# Autodesk Inventor assembly: inner
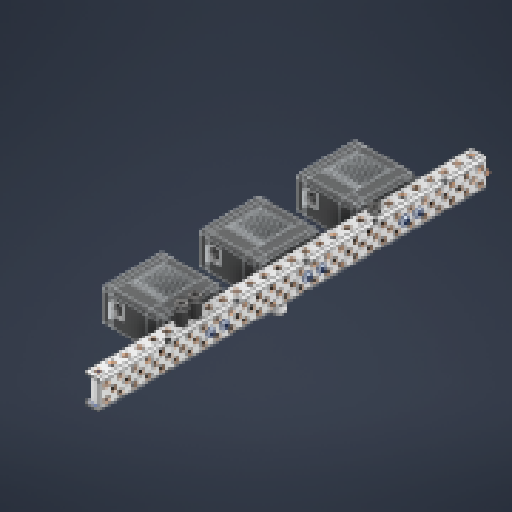
[picture p0: Inventor's stored thumbnail of the model, 512x512]
Saved by Autodesk Inventor 2024 (Build 280153000, 153)
## iProperties
Created: 2023-10-29
Part Number: inner
Document SubType Name: Assembly
Designer: avere
Author: avere
## Documents named in this file (17)
- C:\Users\avere\Documents\rbp_cad\zoomba_v0.1\chassis\drivebay\inner.iam
- C:\Users\avere\Documents\rbp_cad\VEX-CAD-Inventor-1.41\Structure\C Channel\Aluminum 1x2x1\Alu C 1x2x1x28.ipt
- C:\Users\avere\Documents\rbp_cad\VEX-CAD-Inventor-1.41\Electronics\Motors with Screws\SteelM-StarS.iam
- C:\Users\avere\Documents\rbp_cad\VEX-CAD-Inventor-1.41\Electronics\Motors with Screws.iam
- C:\Users\avere\Documents\rbp_cad\hardware\.375 OD Aluminum Spacer 0.875.ipt
- C:\Users\avere\Documents\rbp_cad\VEX-CAD-Inventor-1.41\Motion\Spacers\Spacer Nylon .375 OD.ipt
- C:\Users\avere\Documents\rbp_cad\VEX-CAD-Inventor-1.41\Motion\Spacers\Spacer Nylon .375 OD\NSpacer .375 OD x .500.ipt
- C:\Users\avere\Documents\rbp_cad\zoomba_v0.1\chassis\drivebay\custom_parts\washer_thick.ipt
- C:\Users\avere\Documents\rbp_cad\VEX-CAD-Inventor-1.41\Motion\Spacers\Spacer Nylon .500 OD\NSpacer White .500 OD x .250.ipt
- C:\Users\avere\Documents\rbp_cad\VEX-CAD-Inventor-1.41\Motion\Spacers\Spacer Nylon .500 OD.ipt
- C:\Users\avere\Documents\rbp_cad\VEX-CAD-Inventor-1.41\Structure\Standoff\Standoff .875.ipt
- C:\Users\avere\Documents\rbp_cad\VEX-CAD-Inventor-1.41\Structure\Standoff.ipt
- C:\Users\avere\Documents\rbp_cad\VEX-CAD-Inventor-1.41\Motion\Spacers\Spacer Nylon .375 OD\NSpacer .375 OD x .125.ipt
- C:\Users\avere\Documents\rbp_cad\VEX-CAD-Inventor-1.41\Motion\Spacers\Washer Steel\SWasher .375 OD x .062500.ipt
- C:\Users\avere\Documents\rbp_cad\VEX-CAD-Inventor-1.41\Motion\Spacers\Washer Steel.ipt
- C:\Users\avere\Documents\rbp_cad\VEX-CAD-Inventor-1.41\Motion\Spacers\Washer Steel\SWasher .375 OD x .015625.ipt
- C:\Users\avere\Documents\rbp_cad\VEX-CAD-Inventor-1.41\Motion\Spacers\Washer Steel\SWasher .375 OD x .031250.ipt
## Components (22 placed, 11 different names)
1. Alu C 1x2x1x28:1 — Insert:5, Mate:1, Insert:6, Mate:2, Insert:7, Mate:3, Insert:8, Insert:22, Insert:27, Insert:28, Insert:29, Insert:30, Insert:31, Insert:32, Insert:35, Insert:40, Insert:41
2. SteelM-StarS:1 [sub-assembly] — Insert:5, Mate:1
3. SteelM-StarS:2 [sub-assembly] — Insert:6, Mate:2
4. SteelM-StarS:3 [sub-assembly] — Insert:7, Mate:3
5. .375 OD Aluminum Spacer 0.875:1 — Insert:8
6. washer_thick:1 — Insert:22
7. NSpacer White .500 OD x .250:1
8. Standoff .875:1 — Insert:27
9. Standoff .875:2 — Insert:28
10. Standoff .875:3 — Insert:29
11. Standoff .875:4 — Insert:30
12. Standoff .875:5 — Insert:31
13. .375 OD Aluminum Spacer 0.875:2 — Insert:32
14. NSpacer .375 OD x .125:17 — Insert:35
15. SWasher .375 OD x .062500:1
16. SWasher .375 OD x .015625:2
17. SWasher .375 OD x .031250:3
18. NSpacer .375 OD x .500:18 — Insert:41
19. NSpacer .375 OD x .125:19
20. SWasher .375 OD x .031250:4
21. NSpacer .375 OD x .500:20 — Insert:40
22. NSpacer .375 OD x .125:21
## Relationships (24: Insert 21, Mate 3)
- Insert:5: Alu C 1x2x1x28:1 ↔ SteelM-StarS:1
- Mate:1: Alu C 1x2x1x28:1 ↔ SteelM-StarS:1
- Insert:6: Alu C 1x2x1x28:1 ↔ SteelM-StarS:2
- Mate:2: Alu C 1x2x1x28:1 ↔ SteelM-StarS:2
- Insert:7: Alu C 1x2x1x28:1 ↔ SteelM-StarS:3
- Mate:3: Alu C 1x2x1x28:1 ↔ SteelM-StarS:3
- Insert:8: Alu C 1x2x1x28:1 ↔ .375 OD Aluminum Spacer 0.875:1
- [Insert]: washer_thick:1 ↔ NSpacer White .500 OD x .250:1
- Insert:22: Alu C 1x2x1x28:1 ↔ washer_thick:1
- Insert:27: Alu C 1x2x1x28:1 ↔ Standoff .875:1
- Insert:28: Alu C 1x2x1x28:1 ↔ Standoff .875:2
- Insert:29: Alu C 1x2x1x28:1 ↔ Standoff .875:3
- Insert:30: Alu C 1x2x1x28:1 ↔ Standoff .875:4
- Insert:31: Alu C 1x2x1x28:1 ↔ Standoff .875:5
- Insert:32: Alu C 1x2x1x28:1 ↔ .375 OD Aluminum Spacer 0.875:2
- [Insert]: SWasher .375 OD x .062500:1 ↔ SWasher .375 OD x .015625:2
- [Insert]: NSpacer .375 OD x .125:17 ↔ SWasher .375 OD x .062500:1
- Insert:35: Alu C 1x2x1x28:1 ↔ NSpacer .375 OD x .125:17
- [Insert]: NSpacer .375 OD x .500:18 ↔ NSpacer .375 OD x .125:19
- [Insert]: SWasher .375 OD x .031250:3 ↔ NSpacer .375 OD x .125:19
- [Insert]: NSpacer .375 OD x .500:20 ↔ NSpacer .375 OD x .125:21
- [Insert]: SWasher .375 OD x .031250:4 ↔ NSpacer .375 OD x .125:21
- Insert:40: Alu C 1x2x1x28:1 ↔ NSpacer .375 OD x .500:20
- Insert:41: Alu C 1x2x1x28:1 ↔ NSpacer .375 OD x .500:18
## Named parameters: d40_d23 = 0 mm, d44_d242 = 0 mm, d47_d243 = 0 mm
